# Autodesk Inventor assembly: eccentricWheel
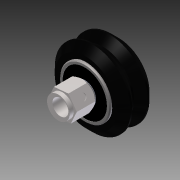
[picture p0: Inventor's stored thumbnail of the model, 180x180]
Saved by Autodesk Inventor 2015 (Build 190159000, 159)
## iProperties
Created: 2013-10-04
Part Number: eccentricWheel
Document SubType Name: Assembly
Designer: Michael
Author: Michael
## Documents named in this file (5)
- C:\Users\Michael\Dropbox\autocad\openbuild\parts\eccentricWheel.iam
- C:\Users\Michael\Dropbox\autocad\openbuild\parts\V-Slot Solid Works\Wheels\Imported Components\ball_bearing\ball_bearing.ipt
- C:\Users\Michael\Dropbox\autocad\openbuild\parts\V-Slot Solid Works\Wheels\Imported Components\dual_v_wheel\dual_v_wheel.ipt
- C:\Users\Michael\Dropbox\autocad\openbuild\parts\10x5x1mmShim.ipt
- C:\Users\Michael\Dropbox\autocad\openbuild\parts\V-Slot Solid Works\Wheels\Imported Components\eccentric_spacer\eccentric_spacer.ipt
## Components (5 placed, 4 different names)
1. ball_bearing:1 — Mate:3, Mate:4, Insert:2
2. dual_v_wheel:1 — Mate:1, Mate:2, Mate:3, Mate:4
3. ball_bearing:2 — Insert:1, Mate:1, Mate:2
4. 10x5x1mmShim:1 — Insert:1
5. eccentric_spacer:1 — Insert:2
## Relationships (6: Mate 4, Insert 2)
- Insert:1: ball_bearing:2 ↔ 10x5x1mmShim:1
- Mate:1: dual_v_wheel:1 ↔ ball_bearing:2
- Mate:2: dual_v_wheel:1 ↔ ball_bearing:2
- Mate:3: ball_bearing:1 ↔ dual_v_wheel:1
- Mate:4: ball_bearing:1 ↔ dual_v_wheel:1
- Insert:2: ball_bearing:1 ↔ eccentric_spacer:1
